# Autodesk Inventor assembly: p80 support post
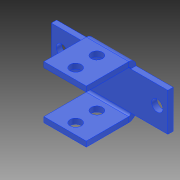
[picture p0: Inventor's stored thumbnail of the model, 180x180]
Saved by Autodesk Inventor 2013 (Build 170138000, 138)
## iProperties
Created: 2013-02-03
Part Number: p80 support post
Document SubType Name: Assembly
Designer: Arpan
Mass: 300.503 g
Surface Area: 752.692 cm^2
Volume: 113.679 cm^3
Density: 2.64343 g/cm^3
Author: Arpan
## Documents named in this file (5)
- C:\Users\Arpan\Documents\GitHub\frc2013CAD\Cimber actual\p80 support post.iam
- C:\Users\Arpan\Documents\GitHub\frc2013CAD\Cimber actual\p80 mount.ipt
- C:\Users\Arpan\Documents\GitHub\frc2013CAD\Cimber actual\Winch mount frange.ipt
- C:\Users\Arpan\Documents\GitHub\frc2013CAD\Cimber actual\p80 bearing mount.ipt
- C:\Users\Arpan\Downloads\Imported Components\6383K234\6383K234.ipt
## Components (4 placed, 4 different names)
1. p80 mount:1 — Mate:1, Mate:2, Mate:3
2. Winch mount frange:1 — Mate:1, Mate:2, Mate:3, Mate:4, Mate:5, Mate:6
3. p80 bearing mount:1 — Mate:4, Mate:5, Mate:6, Mate:7, Mate:8
4. 6383K234:1 — Mate:7, Mate:8
## Relationships (8: Mate 8)
- Mate:1: p80 mount:1 ↔ Winch mount frange:1
- Mate:2: p80 mount:1 ↔ Winch mount frange:1
- Mate:3: p80 mount:1 ↔ Winch mount frange:1
- Mate:4: Winch mount frange:1 ↔ p80 bearing mount:1
- Mate:5: Winch mount frange:1 ↔ p80 bearing mount:1
- Mate:6: Winch mount frange:1 ↔ p80 bearing mount:1
- Mate:7: p80 bearing mount:1 ↔ 6383K234:1
- Mate:8: p80 bearing mount:1 ↔ 6383K234:1
